# Autodesk Inventor assembly: AddOn_Module
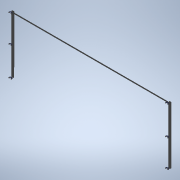
[picture p0: Inventor's stored thumbnail of the model, 180x180]
Saved by Autodesk Inventor 2021 (Build 250183000, 183)
## iProperties
Created: 2021-04-05
Part Number: AddOn_Module
Document SubType Name: Assembly
Designer: Jorian Brusind
Author: Jorian Brusind
## Documents named in this file (5)
- C:\Users\Jorian Bruslind\Documents\GitHub\PersonalProjects\HyperRail\Inventor Files\AddOn_Module.iam
- C:\Users\Jorian Bruslind\Documents\GitHub\PersonalProjects\Inventor Projects\Useful models\8020_Sets\IPT_40_Series\Extra_40_Series\HFS5-4060-4000\HFS5-4060-2125.ipt
- C:\Users\Jorian Bruslind\Documents\GitHub\PersonalProjects\HyperRail\Inventor Files\SDP_sdpsi_a_6r25mc250\SDP_sdpsi_a_6r25mc1000.ipt
- C:\Users\Jorian Bruslind\Documents\GitHub\PersonalProjects\HyperRail\Inventor Files\SpacingStrut.iam
- C:\Users\Jorian Bruslind\Documents\GitHub\PersonalProjects\HyperRail\Inventor Files\Bottom_Foot_Assembly.iam
## Components (13 placed, 4 different names)
1. HFS5-4060-2125:1 — Mate:35, Flush:40, Mate:59, Mate:60, Flush:43, Mate:62, Mate:63, Flush:52, Flush:53, Flush:54
2. SDP_sdpsi_a_6r25mc1000:1
3. SDP_sdpsi_a_6r25mc1000:2
4. HFS5-4060-2125:2 — Flush:40, Mate:60, Flush:41, Mate:61, Mate:65, Mate:66, Flush:55, Flush:56
5. SDP_sdpsi_a_6r25mc1000:3
6. SDP_sdpsi_a_6r25mc1000:4
7. SpacingStrut:1 [sub-assembly] — Mate:59, Flush:41, Mate:61, Flush:43, Mate:62
8. Bottom_Foot_Assembly:1 [sub-assembly] — Flush:47, Flush:48, Flush:49, Flush:56, Mate:67
9. Bottom_Foot_Assembly:2 [sub-assembly] — Flush:46, Flush:48, Mate:67
10. Bottom_Foot_Assembly:3 [sub-assembly] — Flush:46, Flush:47, Flush:49, Mate:65, Mate:66, Flush:55
11. Bottom_Foot_Assembly:4 [sub-assembly] — Flush:45, Flush:50, Flush:51, Flush:53
12. Bottom_Foot_Assembly:5 [sub-assembly] — Flush:44, Flush:50, Flush:52, Flush:54, Mate:64
13. Bottom_Foot_Assembly:6 [sub-assembly] — Flush:44, Flush:45, Flush:51, Mate:63, Mate:64
## Relationships (38: Flush 24, Mate 14)
- [Flush]: SDP_sdpsi_a_6r25mc1000:1 ↔ SDP_sdpsi_a_6r25mc1000:2
- [Mate]: SDP_sdpsi_a_6r25mc1000:1 ↔ SDP_sdpsi_a_6r25mc1000:2
- [Flush]: SDP_sdpsi_a_6r25mc1000:1 ↔ SDP_sdpsi_a_6r25mc1000:2
- [Mate] (1 mm): HFS5-4060-2125:1 ↔ SDP_sdpsi_a_6r25mc1000:1
- [Flush]: HFS5-4060-2125:1 ↔ SDP_sdpsi_a_6r25mc1000:1
- [Flush]: HFS5-4060-2125:1 ↔ SDP_sdpsi_a_6r25mc1000:1
- Mate:35: HFS5-4060-2125:1
- [Flush]: SDP_sdpsi_a_6r25mc1000:3 ↔ SDP_sdpsi_a_6r25mc1000:4
- [Mate]: SDP_sdpsi_a_6r25mc1000:3 ↔ SDP_sdpsi_a_6r25mc1000:4
- [Flush]: SDP_sdpsi_a_6r25mc1000:3 ↔ SDP_sdpsi_a_6r25mc1000:4
- [Mate] (1 mm): HFS5-4060-2125:2 ↔ SDP_sdpsi_a_6r25mc1000:3
- [Flush]: HFS5-4060-2125:2 ↔ SDP_sdpsi_a_6r25mc1000:3
- [Flush]: HFS5-4060-2125:2 ↔ SDP_sdpsi_a_6r25mc1000:3
- Flush:40: HFS5-4060-2125:1 ↔ HFS5-4060-2125:2
- Mate:59 (-20 mm): HFS5-4060-2125:1 ↔ SpacingStrut:1
- Mate:60 (5793 mm): HFS5-4060-2125:1 ↔ HFS5-4060-2125:2
- Flush:41: HFS5-4060-2125:2 ↔ SpacingStrut:1
- Mate:61: HFS5-4060-2125:2 ↔ SpacingStrut:1
- Flush:43: HFS5-4060-2125:1 ↔ SpacingStrut:1
- Mate:62: HFS5-4060-2125:1 ↔ SpacingStrut:1
- Flush:44: Bottom_Foot_Assembly:5 ↔ Bottom_Foot_Assembly:6
- Flush:45: Bottom_Foot_Assembly:4 ↔ Bottom_Foot_Assembly:6
- Flush:46: Bottom_Foot_Assembly:2 ↔ Bottom_Foot_Assembly:3
- Flush:47: Bottom_Foot_Assembly:1 ↔ Bottom_Foot_Assembly:3
- Flush:48: Bottom_Foot_Assembly:1 ↔ Bottom_Foot_Assembly:2
- Flush:49: Bottom_Foot_Assembly:1 ↔ Bottom_Foot_Assembly:3
- Flush:50: Bottom_Foot_Assembly:4 ↔ Bottom_Foot_Assembly:5
- Flush:51: Bottom_Foot_Assembly:4 ↔ Bottom_Foot_Assembly:6
- Mate:63: HFS5-4060-2125:1 ↔ Bottom_Foot_Assembly:6
- Flush:52 (20 mm): HFS5-4060-2125:1 ↔ Bottom_Foot_Assembly:5
- Flush:53: HFS5-4060-2125:1 ↔ Bottom_Foot_Assembly:4
- Flush:54: HFS5-4060-2125:1 ↔ Bottom_Foot_Assembly:5
- Mate:64 (1000 mm): Bottom_Foot_Assembly:5 ↔ Bottom_Foot_Assembly:6
- Mate:65: HFS5-4060-2125:2 ↔ Bottom_Foot_Assembly:3
- Mate:66 (-20 mm): HFS5-4060-2125:2 ↔ Bottom_Foot_Assembly:3
- Flush:55: HFS5-4060-2125:2 ↔ Bottom_Foot_Assembly:3
- Flush:56: HFS5-4060-2125:2 ↔ Bottom_Foot_Assembly:1
- Mate:67 (1000 mm): Bottom_Foot_Assembly:1 ↔ Bottom_Foot_Assembly:2
## Named parameters: d97_d633 = 0 mm, d98_d634 = 0 mm, d99_d635 = 0 mm, d100_d636 = 1 mm, d101_d637 = 0 mm, d102_d638 = 0 mm
